# Autodesk Inventor assembly: Assembly2
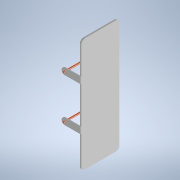
[picture p0: Inventor's stored thumbnail of the model, 180x180]
Saved by Autodesk Inventor 2022.2 (Build 262287000, 287)
## iProperties
Created: 2022-02-27
Part Number: Assembly2
Document SubType Name: Assembly
Designer: PRASHANTH
Author: PRASHANTH
## Documents named in this file (4)
- E:\BME\Autodesk Sample\Engg Exploration\Subsystem1-Conveyor Belt\Assembly2.iam
- E:\BME\Autodesk Sample\Engg Exploration\Subsystem1-Conveyor Belt\Conveyor Base.ipt
- E:\BME\Autodesk Sample\Engg Exploration\Subsystem1-Conveyor Belt\Conveyor Stand.ipt
- E:\BME\Autodesk Sample\Engg Exploration\Subsystem1-Conveyor Belt\Conveyor Shaft Pin.ipt
## Components (5 placed, 3 different names)
1. Conveyor Base:1 — Mate:1, Mate:2, Flush:1, Flush:2
2. Conveyor Stand:1 — Insert:2, Mate:2, Flush:1
3. Conveyor Stand:2 — Insert:1, Mate:1, Flush:2
4. Conveyor Shaft Pin:1 — Insert:1
5. Conveyor Shaft Pin:2 — Insert:2
## Relationships (6: Insert 2, Mate 2, Flush 2)
- Insert:1 (-5 mm): Conveyor Stand:2 ↔ Conveyor Shaft Pin:1
- Insert:2 (-5 mm): Conveyor Stand:1 ↔ Conveyor Shaft Pin:2
- Mate:1: Conveyor Base:1 ↔ Conveyor Stand:2
- Mate:2: Conveyor Base:1 ↔ Conveyor Stand:1
- Flush:1: Conveyor Base:1 ↔ Conveyor Stand:1
- Flush:2: Conveyor Base:1 ↔ Conveyor Stand:2
